# Autodesk Inventor assembly: LHSA 10
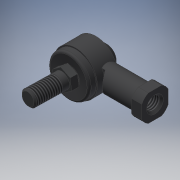
[picture p0: Inventor's stored thumbnail of the model, 180x180]
Saved by Autodesk Inventor 2018 (Build 220112000, 112)
## iProperties
Category: PARTsolutions
Company: IKO
Created: 2017-10-01
Part Number: LHSA 10
Catalog Web Link: www.cadenas.de
Description: LHSA-
Vendor: IKO
Document SubType Name: Assembly
Designer: psAdmin
Manufacturer: IKO
PSOL_IDENT_0: {$CADENAS_DATA\23d-libs\iko\iko_bearings\l_balls\lhsa_1_asmtab.prj},159 {VTYP=3D},{STYP=ASSTAB},{NB=
PSOL_IDENT_1: LHSA 10},{LINA=LHSA 10},{NN=LHSA},{DATE=13.10.2016 10:02:12},{GEOMDATE=03.01.2008},{VERSION=},{LINEI
PSOL_IDENT_2: D=60},{LINESUBID=-1},{WBVAR=}  {NB=LHSA 10},{LINA=LHSA 10},{KT=DUMMY},{IDNR=},{ORDER=LHSA 10},{RID=G
PSOL_IDENT_3: _50},{STDRT=10},{DESCR=LHSA},{TRNUMBER=},{PAST=A},{REST=O},{MASS=106},{S=M10x1.25},{KDM=8.466},{NDM=
PSOL_IDENT_4: 10.000},{P1=1.250},{V=10},{D=28},{L=57.0},{L1=43},{L2=23},{SL1=6.5},{W=17},{W1=17},{W2=17},{D1=15.0}
PSOL_IDENT_5: ,{D2=19},{LL=49.0},{P=12.0},{LL1=16.0},{LL2=21.0},{LL3=17.0},{SDK=19.050},{V1=11.0},{D3=12.2475},{D4=
PSOL_IDENT_6: 21.2001},{D5=26.3},{D6=25.65},{L3=53.8825},{L4=26.1906},{L5=28.5},{L12=30.1645},{B=8.5},{B1=5.0},{B2=
PSOL_IDENT_7: 6.5},{B3=11.5},{B4=13.0},{B5=17.5073},{LL4=4.5},{LL5=9.0},{CB=0.0},{CC=0.9},{E=0},{F=0.0},{C1=1.1765
PSOL_IDENT_8: },{C2=1.0},{R1=5},{R2=34.5114},{R3=15.7},{R4=1.3},{CS=7400},{SS1=8.160},{S1=10},{LX=25},{LX1=28.0},{
PSOL_IDENT_9: BL=3},{SC=1},{PPATH=lhsa_1_asmtpl.prj}
NN: LHSA
NB: LHSA 10
NBSYN: $ORDER.
LINA: LHSA 10
ORDER: LHSA 10
MASS: 106
S: M10x1.25
V: 10
D: 28
L: 57.0
L1: 43
L2: 23
SL1: 6.5
W1: 17
W2: 17
D1: 15.0
D2: 19
LL: 49.0
P: 12.0
LL1: 16.0
LL2: 21.0
LL3: 17.0
SDK: 19.050
CS: 7400
SUPPLIER: IKO
ARTICLENO: LHSA 10
BOMINFO: LHSA 10
CREATOR: CADENAS GmbH
Title: LHSA 10
Author: Cadenas PARTsolutions
## Documents named in this file (3)
- C:\Users\mura5\Documents\RBBR\cart\前足改\ステア\AIS2016\LHSA 10.iam
- C:\Users\mura5\Documents\RBBR\cart\前足改\ステア\AIS2016\LHSA 10 Body2.ipt
- C:\Users\mura5\Documents\RBBR\cart\前足改\ステア\AIS2016\LHSA 10 Body1.ipt
## Components (2 placed, 2 different names)
1. LHSA 10 Body2:1 — ボール:1
2. LHSA 10 Body1:1 — ボール:1
## Relationships (1: BallJoint 1)
- ボール:1 [BallJoint]: LHSA 10 Body2:1 ↔ LHSA 10 Body1:1
